# Autodesk Inventor assembly: ASM
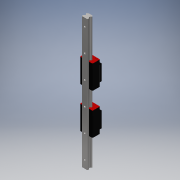
[picture p0: Inventor's stored thumbnail of the model, 180x180]
Saved by Autodesk Inventor 2016 (Build 200138000, 138)
## iProperties
Created: 2017-01-18
Part Number: ASM
Material: Типовые
Document SubType Name: Assembly
Designer: stan
Author: stan
## Documents named in this file (4)
- C:\Users\stan\Documents\Inventor\SELVOX-1500\Z\ASM.iam
- ASM.iam
- C:\Users\stan\Documents\Inventor\SELVOX-1500\Z\[Z] HGR15R.ipt
- C:\Users\stan\Documents\Inventor\SELVOX-1500\Z\[Z] HGH15CA.ipt
## Components (3 placed, 2 different names)
1. [Z] HGR15R:1 — Ползун:1, Ползун:2
2. [Z] HGH15CA:1 — Ползун:1
3. [Z] HGH15CA:2 — Ползун:2
## Relationships (2: TranslationJoint 2)
- Ползун:1 [TranslationJoint]: [Z] HGR15R:1 ↔ [Z] HGH15CA:1
- Ползун:2 [TranslationJoint]: [Z] HGR15R:1 ↔ [Z] HGH15CA:2
